# Autodesk Inventor assembly: Assembly1
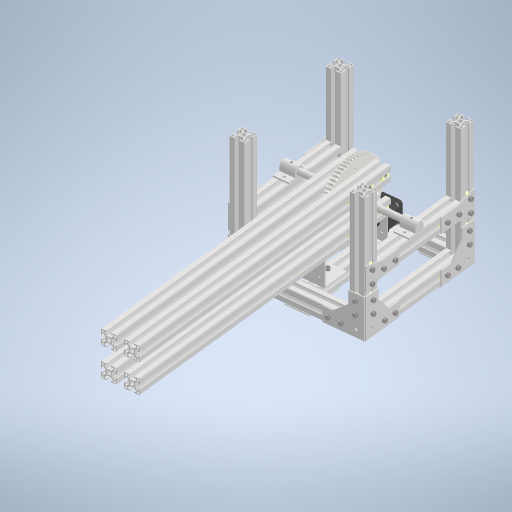
[picture p0: Inventor's stored thumbnail of the model, 512x512]
Saved by Autodesk Inventor 2024 (Build 280153000, 153)
## iProperties
Created: 2025-12-08
Part Number: Assembly1
Document SubType Name: Assembly
Designer: schar
Author: schar
## Documents named in this file (22)
- C:\Users\schar\Desktop\projectBlueprint\AMSTS\hardware\Assembly1.iam
- C:\Users\schar\Desktop\projectBlueprint\AMSTS\hardware\3030_200.ipt
- C:\Users\schar\Desktop\projectBlueprint\AMSTS\hardware\Connect2x3030_m6.ipt
- C:\Users\schar\Desktop\projectBlueprint\AMSTS\hardware\3030_tnut_m6.ipt
- C:\Users\schar\Documents\Inventor\Content Center Files\R2024\en-US\AS 1420\AS 1420 - 1973 - M5 x 10.ipt
- C:\Users\schar\Desktop\projectBlueprint\AMSTS\hardware\3030_260.ipt
- C:\Users\schar\Desktop\projectBlueprint\AMSTS\hardware\3030_connector_assembled.iam
- C:\Users\schar\Desktop\projectBlueprint\AMSTS\hardware\3030_connector_assembled_MIR.iam
- C:\Users\schar\Desktop\projectBlueprint\AMSTS\hardware\3030_connector_assembled_MIR1.iam
- C:\Users\schar\Desktop\projectBlueprint\AMSTS\hardware\3030_connector_assembled_MIR_MIR.iam
- C:\Users\schar\Desktop\projectBlueprint\AMSTS\hardware\3030_T_connector_assembled.iam
- C:\Users\schar\Desktop\projectBlueprint\AMSTS\hardware\3030_T_connector_assembled_MIR1.iam
- C:\Users\schar\Desktop\projectBlueprint\AMSTS\hardware\NEMA 17 - MS17HD2.iam
- C:\Users\schar\Desktop\projectBlueprint\AMSTS\hardware\wormgear_pol_base.iam
- C:\Users\schar\Desktop\projectBlueprint\AMSTS\hardware\base_axis_static_12mm.ipt
- C:\Users\schar\Desktop\projectBlueprint\AMSTS\hardware\base_axis_12mm.ipt
- C:\Users\schar\Desktop\projectBlueprint\AMSTS\hardware\NEMA17-3030-m6-holder.ipt
- C:\Users\schar\Desktop\projectBlueprint\AMSTS\hardware\3030_tnut_m6_main.ipt
- C:\Users\schar\Desktop\projectBlueprint\AMSTS\hardware\basis-bearing-3030-m6-holder.ipt
- C:\Users\schar\Desktop\projectBlueprint\AMSTS\hardware\wormgear_axis_6mm.ipt
- C:\Users\schar\Desktop\projectBlueprint\AMSTS\hardware\wormgear_worm_axes_holder.ipt
- C:\Users\schar\Desktop\projectBlueprint\AMSTS\hardware\Az_rot_3030_with_holes.ipt
## Components (94 placed, 21 different names)
1. 3030_tnut_m6_main:1 — Rotational:16
2. 3030_tnut_m6_main:2 — Rigid:3
3. 3030_tnut_m6_main:3 — Rotational:17, Flush:34
4. 3030_tnut_m6_main:4 — Rotational:18
5. wormgear_axis_6mm:1 — Mate:61, Mate:62, Mate:63, Mate:64, Mate:65
6. wormgear_worm_axes_holder:1 — Mate:64, Mate:65
7. Az_rot_3030_with_holes:1 — Mate:66, Mate:67, Mate:68, Mate:84, Mate:85, Mate:86, Mate:87, Mate:88, Mate:89
8. Az_rot_3030_with_holes:2 — Mate:75, Mate:76, Mate:77, Mate:90, Mate:91, Mate:92, Mate:93, Mate:94, Mate:95
9. Az_rot_3030_with_holes:3 — Mate:69, Mate:70, Mate:71, Mate:78, Mate:79, Mate:80, Mate:81, Mate:82, Mate:83
10. Az_rot_3030_with_holes:4 — Mate:72, Mate:73, Mate:74, Mate:96, Mate:97, Mate:98, Mate:99, Mate:100, Mate:101
11. 3030_tnut_m6_main:5 — Mate:80, Mate:81
12. 3030_tnut_m6_main:6 — Mate:82, Mate:83
13. 3030_tnut_m6_main:7 — Mate:84, Mate:87
14. 3030_tnut_m6_main:8 — Mate:78, Mate:79
15. 3030_tnut_m6_main:9 — Mate:85, Mate:88
16. 3030_tnut_m6_main:10 — Mate:86, Mate:89
17. 3030_tnut_m6_main:11 — Mate:96, Mate:97
18. 3030_tnut_m6_main:12 — Mate:99, Mate:101
19. 3030_tnut_m6_main:13 — Mate:98, Mate:100
20. 3030_tnut_m6_main:14 — Mate:90, Mate:92
21. 3030_tnut_m6_main:15 — Mate:91, Mate:93
22. 3030_tnut_m6_main:16 — Mate:94, Mate:95
23. 3030_200:1 — Mate:1, Mate:2, Flush:1, Flush:2, Mate:4, Flush:5, Flush:6, Symmetry:1, Mate:30, Mate:45, Flush:18, Mate:48
24. 3030_200:2 — Mate:3, Flush:3, Flush:4, Mate:6, Flush:9, Flush:10, Symmetry:2
25. Connect2x3030_m6:1 — Mate:1, Mate:2, Flush:1, Flush:2, Mate:3, Flush:3, Flush:4, Rigid:1, Rotational:5, Rotational:6, Rotational:7, Insert:11, Insert:12, Insert:14, Insert:15, Mate:19, Mate:20, Mate:21, Mate:36, Mate:37
26. Connect2x3030_m6:2 — Mate:4, Flush:5, Flush:6, Mate:5, Flush:7, Flush:8, Rotational:1, Rotational:2, Rotational:3, Rotational:4, Insert:6, Insert:7, Insert:9, Insert:10, Mate:10, Mate:11, Mate:12, Mate:32, Mate:33
27. Connect2x3030_m6:3 — Mate:8, Flush:11, Flush:12, Rotational:12, Rotational:13, Rotational:14, Rotational:15, Insert:1, Insert:2, Insert:4, Insert:5, Mate:13, Mate:14, Mate:15, Mate:40, Mate:41
28. Connect2x3030_m6:4 — Mate:6, Flush:9, Flush:10, Mate:7, Flush:13, Mate:9, Flush:14, Rotational:8, Rotational:9, Rotational:10, Rotational:11, Insert:16, Insert:17, Insert:18, Insert:20, Mate:16, Mate:17, Mate:18, Mate:23, Flush:15, Mate:25
29. 3030_200:3 — Mate:5, Flush:7, Flush:8, Mate:8, Flush:11, Flush:12, Symmetry:2, Mate:52
30. 3030_200:4 — Flush:13, Mate:9, Flush:14, Symmetry:1, Mate:53, Flush:23
31. 3030_connector_assembled:1 [sub-assembly] — Mate:24, Mate:25, Mate:26
32. 3030_connector_assembled:2 [sub-assembly] — Mate:22, Mate:23, Flush:15, Mate:26
33. 3030_connector_assembled_MIR:1 [sub-assembly] — Mate:27, Mate:39, Mate:40
34. 3030_connector_assembled_MIR:2 [sub-assembly] — Mate:27, Mate:38, Mate:41
35. 3030_connector_assembled_MIR1:1 [sub-assembly] — Mate:28, Mate:34, Mate:37
36. 3030_connector_assembled_MIR1:2 [sub-assembly] — Mate:28, Mate:35, Mate:36
37. 3030_connector_assembled_MIR_MIR:1 [sub-assembly] — Mate:29, Mate:30, Mate:33
38. 3030_connector_assembled_MIR_MIR:2 [sub-assembly] — Mate:29, Mate:31, Mate:32
39. 3030_260:1 — Mate:10, Mate:11, Mate:12, Mate:31, Mate:49, Flush:20
40. 3030_260:2 — Mate:13, Mate:14, Mate:15, Mate:38, Mate:39, Mate:42, Flush:16
41. 3030_260:3 — Mate:16, Mate:17, Mate:18, Mate:22, Mate:24, Mate:43, Flush:17
42. 3030_260:4 — Mate:19, Mate:20, Mate:21, Mate:34, Mate:35, Mate:50, Flush:21
43. NEMA 17 - MS17HD2:1 [sub-assembly] — Rotational:19, Rotational:20, Mate:61, Mate:62
44. wormgear_pol_base:1 [sub-assembly] — Rigid:2, Mate:63, Mate:66, Mate:67, Mate:68, Mate:69, Mate:70, Mate:71, Mate:72, Mate:73, Mate:74, Mate:75, Mate:76, Mate:77
45. base_axis_static_12mm:1 — Flush:30, Mate:57, Insert:22
46. base_axis_static_12mm:2 — Mate:58, Flush:31, Flush:32, Insert:21
47. base_axis_12mm:1 — Insert:21, Insert:22, Rigid:2
48. basis-bearing-3030-m6-holder:1 — Mate:60, Flush:35, Rotational:18, Flush:36, Rigid:3, Insert:23, Insert:24
49. NEMA17-3030-m6-holder:1 — Mate:59, Flush:33, Rotational:16, Rotational:17, Insert:25, Insert:26, Rotational:19, Rotational:20
50. 3030_T_connector_assembled:1 [sub-assembly] — Mate:43, Flush:17, Mate:56, Flush:29
51. 3030_T_connector_assembled:2 [sub-assembly] — Mate:42, Flush:16, Flush:26
52. 3030_T_connector_assembled_MIR1:1 [sub-assembly] — Mate:50, Flush:21, Mate:55, Flush:27, Flush:28
53. 3030_T_connector_assembled_MIR1:2 [sub-assembly] — Mate:49, Flush:20, Mate:54, Flush:24, Flush:25
54. 3030_T_connector_assembled:3 [sub-assembly] — Mate:45, Flush:18, Mate:47, Flush:19
55. 3030_200:5 — Mate:47, Mate:48, Flush:19, Mate:52, Flush:22, Mate:59, Flush:33, Flush:34, Mate:60, Flush:35, Flush:36
56. 3030_T_connector_assembled:4 [sub-assembly] — Mate:53, Flush:22, Flush:23
57. 3030_200:6 — Mate:55, Flush:27, Flush:28, Mate:56, Flush:29, Flush:30, Mate:57
58. 3030_200:7 — Mate:54, Flush:24, Flush:25, Flush:26, Mate:58, Flush:31, Flush:32
59. 3030_tnut_m6:1 — Rotational:12
60. 3030_tnut_m6:2 — Rotational:11
61. 3030_tnut_m6:3 — Rigid:1
62. 3030_tnut_m6:4 — Rotational:1
63. 3030_tnut_m6:5 — Rotational:13
64. 3030_tnut_m6:6 — Rotational:10
65. 3030_tnut_m6:7 — Rotational:5
66. 3030_tnut_m6:8 — Rotational:2
67. 3030_tnut_m6:9 — Rotational:15
68. 3030_tnut_m6:10 — Rotational:8
69. 3030_tnut_m6:11 — Rotational:6
70. 3030_tnut_m6:12 — Rotational:4
71. 3030_tnut_m6:13 — Rotational:14
72. 3030_tnut_m6:14 — Rotational:9
73. 3030_tnut_m6:15 — Rotational:7
74. 3030_tnut_m6:16 — Rotational:3
75. AS 1420 - Metric M5 x 10:1 — Insert:1
76. AS 1420 - Metric M5 x 10:2 — Insert:2
77. AS 1420 - Metric M5 x 10:4 — Insert:4
78. AS 1420 - Metric M5 x 10:5 — Insert:5
79. AS 1420 - Metric M5 x 10:6 — Insert:6
80. AS 1420 - Metric M5 x 10:7 — Insert:7
81. AS 1420 - Metric M5 x 10:9 — Insert:9
82. AS 1420 - Metric M5 x 10:10 — Insert:10
83. AS 1420 - Metric M5 x 10:11 — Insert:11
84. AS 1420 - Metric M5 x 10:12 — Insert:12
85. AS 1420 - Metric M5 x 10:14 — Insert:14
86. AS 1420 - Metric M5 x 10:15 — Insert:15
87. AS 1420 - Metric M5 x 10:16 — Insert:16
88. AS 1420 - Metric M5 x 10:17 — Insert:17
89. AS 1420 - Metric M5 x 10:18 — Insert:18
90. AS 1420 - Metric M5 x 10:20 — Insert:20
91. AS 1420 - Metric M5 x 10:21 — Insert:23
92. AS 1420 - Metric M5 x 10:22 — Insert:24
93. AS 1420 - Metric M5 x 10:23 — Insert:25
94. AS 1420 - Metric M5 x 10:24 — Insert:26
## Relationships (181: Mate 98, Flush 36, Insert 22, RevoluteJoint 20, WeldJoint 3, Symmetry 2)
- Mate:1: 3030_200:1 ↔ Connect2x3030_m6:1
- Mate:2: 3030_200:1 ↔ Connect2x3030_m6:1
- Flush:1: 3030_200:1 ↔ Connect2x3030_m6:1
- Flush:2 (30 mm): 3030_200:1 ↔ Connect2x3030_m6:1
- Mate:3: 3030_200:2 ↔ Connect2x3030_m6:1
- Flush:3 (30 mm): 3030_200:2 ↔ Connect2x3030_m6:1
- Flush:4: 3030_200:2 ↔ Connect2x3030_m6:1
- Mate:4: 3030_200:1 ↔ Connect2x3030_m6:2
- Flush:5 (-30 mm): 3030_200:1 ↔ Connect2x3030_m6:2
- Flush:6: 3030_200:1 ↔ Connect2x3030_m6:2
- Mate:5: Connect2x3030_m6:2 ↔ 3030_200:3
- Flush:7 (30 mm): Connect2x3030_m6:2 ↔ 3030_200:3
- Flush:8: Connect2x3030_m6:2 ↔ 3030_200:3
- Mate:6: 3030_200:2 ↔ Connect2x3030_m6:4
- Flush:9 (-30 mm): 3030_200:2 ↔ Connect2x3030_m6:4
- Flush:10: 3030_200:2 ↔ Connect2x3030_m6:4
- Mate:7: Connect2x3030_m6:4
- Mate:8: Connect2x3030_m6:3 ↔ 3030_200:3
- Flush:11 (-30 mm): Connect2x3030_m6:3 ↔ 3030_200:3
- Flush:12: Connect2x3030_m6:3 ↔ 3030_200:3
- Flush:13: Connect2x3030_m6:4 ↔ 3030_200:4
- Mate:9: Connect2x3030_m6:4 ↔ 3030_200:4
- Flush:14 (-30 mm): Connect2x3030_m6:4 ↔ 3030_200:4
- Rotational:1 [RevoluteJoint] (-0.357 mm): Connect2x3030_m6:2 ↔ 3030_tnut_m6:4
- Rotational:2 [RevoluteJoint] (-0.357 mm): Connect2x3030_m6:2 ↔ 3030_tnut_m6:8
- Rotational:3 [RevoluteJoint] (-0.357 mm): Connect2x3030_m6:2 ↔ 3030_tnut_m6:16
- Rotational:4 [RevoluteJoint] (-0.357 mm): Connect2x3030_m6:2 ↔ 3030_tnut_m6:12
- Rigid:1 [WeldJoint] (-0.357 mm): Connect2x3030_m6:1 ↔ 3030_tnut_m6:3
- Rotational:5 [RevoluteJoint] (-0.357 mm): Connect2x3030_m6:1 ↔ 3030_tnut_m6:7
- Rotational:6 [RevoluteJoint] (-0.357 mm): Connect2x3030_m6:1 ↔ 3030_tnut_m6:11
- Rotational:7 [RevoluteJoint] (-0.357 mm): Connect2x3030_m6:1 ↔ 3030_tnut_m6:15
- Rotational:8 [RevoluteJoint] (-0.357 mm): Connect2x3030_m6:4 ↔ 3030_tnut_m6:10
- Rotational:9 [RevoluteJoint] (-0.357 mm): Connect2x3030_m6:4 ↔ 3030_tnut_m6:14
- Rotational:10 [RevoluteJoint] (-0.357 mm): Connect2x3030_m6:4 ↔ 3030_tnut_m6:6
- Rotational:11 [RevoluteJoint] (-0.357 mm): Connect2x3030_m6:4 ↔ 3030_tnut_m6:2
- Rotational:12 [RevoluteJoint] (-0.357 mm): Connect2x3030_m6:3 ↔ 3030_tnut_m6:1
- Rotational:13 [RevoluteJoint]: Connect2x3030_m6:3 ↔ 3030_tnut_m6:5
- Rotational:14 [RevoluteJoint] (-0.357 mm): Connect2x3030_m6:3 ↔ 3030_tnut_m6:13
- Rotational:15 [RevoluteJoint] (-0.357 mm): Connect2x3030_m6:3 ↔ 3030_tnut_m6:9
- Insert:1: Connect2x3030_m6:3 ↔ AS 1420 - Metric M5 x 10:1
- Insert:2: Connect2x3030_m6:3 ↔ AS 1420 - Metric M5 x 10:2
- Insert:4: Connect2x3030_m6:3 ↔ AS 1420 - Metric M5 x 10:4
- Insert:5: Connect2x3030_m6:3 ↔ AS 1420 - Metric M5 x 10:5
- Insert:6: Connect2x3030_m6:2 ↔ AS 1420 - Metric M5 x 10:6
- Insert:7: Connect2x3030_m6:2 ↔ AS 1420 - Metric M5 x 10:7
- Insert:9: Connect2x3030_m6:2 ↔ AS 1420 - Metric M5 x 10:9
- Insert:10: Connect2x3030_m6:2 ↔ AS 1420 - Metric M5 x 10:10
- Insert:11: Connect2x3030_m6:1 ↔ AS 1420 - Metric M5 x 10:11
- Insert:12: Connect2x3030_m6:1 ↔ AS 1420 - Metric M5 x 10:12
- Insert:14: Connect2x3030_m6:1 ↔ AS 1420 - Metric M5 x 10:14
- Insert:15: Connect2x3030_m6:1 ↔ AS 1420 - Metric M5 x 10:15
- Insert:16: Connect2x3030_m6:4 ↔ AS 1420 - Metric M5 x 10:16
- Insert:17: Connect2x3030_m6:4 ↔ AS 1420 - Metric M5 x 10:17
- Insert:18: Connect2x3030_m6:4 ↔ AS 1420 - Metric M5 x 10:18
- Insert:20: Connect2x3030_m6:4 ↔ AS 1420 - Metric M5 x 10:20
- Mate:10: Connect2x3030_m6:2 ↔ 3030_260:1
- Mate:11: Connect2x3030_m6:2 ↔ 3030_260:1
- Mate:12: Connect2x3030_m6:2 ↔ 3030_260:1
- Mate:13: Connect2x3030_m6:3 ↔ 3030_260:2
- Mate:14: Connect2x3030_m6:3 ↔ 3030_260:2
- Mate:15: Connect2x3030_m6:3 ↔ 3030_260:2
- Mate:16: Connect2x3030_m6:4 ↔ 3030_260:3
- Mate:17: Connect2x3030_m6:4 ↔ 3030_260:3
- Mate:18: Connect2x3030_m6:4 ↔ 3030_260:3
- Mate:19: Connect2x3030_m6:1 ↔ 3030_260:4
- Mate:20: Connect2x3030_m6:1 ↔ 3030_260:4
- Mate:21: Connect2x3030_m6:1 ↔ 3030_260:4
- Symmetry:1: 3030_200:1 ↔ 3030_200:4
- Mate:22: 3030_connector_assembled:2 ↔ 3030_260:3
- Mate:23: Connect2x3030_m6:4 ↔ 3030_connector_assembled:2
- Flush:15: Connect2x3030_m6:4 ↔ 3030_connector_assembled:2
- Mate:24: 3030_connector_assembled:1 ↔ 3030_260:3
- Mate:25: Connect2x3030_m6:4 ↔ 3030_connector_assembled:1
- Mate:26: 3030_connector_assembled:1 ↔ 3030_connector_assembled:2
- Symmetry:2: 3030_200:2 ↔ 3030_200:3
- Mate:27: 3030_connector_assembled_MIR:1 ↔ 3030_connector_assembled_MIR:2
- Mate:28: 3030_connector_assembled_MIR1:1 ↔ 3030_connector_assembled_MIR1:2
- Mate:29: 3030_connector_assembled_MIR_MIR:1 ↔ 3030_connector_assembled_MIR_MIR:2
- Mate:30: 3030_200:1 ↔ 3030_connector_assembled_MIR_MIR:1
- Mate:31: 3030_connector_assembled_MIR_MIR:2 ↔ 3030_260:1
- Mate:32: Connect2x3030_m6:2 ↔ 3030_connector_assembled_MIR_MIR:2
- Mate:33: Connect2x3030_m6:2 ↔ 3030_connector_assembled_MIR_MIR:1
- Mate:34: 3030_connector_assembled_MIR1:1 ↔ 3030_260:4
- Mate:35: 3030_connector_assembled_MIR1:2 ↔ 3030_260:4
- Mate:36: Connect2x3030_m6:1 ↔ 3030_connector_assembled_MIR1:2
- Mate:37: Connect2x3030_m6:1 ↔ 3030_connector_assembled_MIR1:1
- Mate:38: 3030_connector_assembled_MIR:2 ↔ 3030_260:2
- Mate:39: 3030_connector_assembled_MIR:1 ↔ 3030_260:2
- Mate:40: Connect2x3030_m6:3 ↔ 3030_connector_assembled_MIR:1
- Mate:41: Connect2x3030_m6:3 ↔ 3030_connector_assembled_MIR:2
- Mate:42: 3030_260:2 ↔ 3030_T_connector_assembled:2
- Flush:16: 3030_260:2 ↔ 3030_T_connector_assembled:2
- Mate:43: 3030_260:3 ↔ 3030_T_connector_assembled:1
- Flush:17: 3030_260:3 ↔ 3030_T_connector_assembled:1
- Mate:45: 3030_200:1 ↔ 3030_T_connector_assembled:3
- Flush:18: 3030_200:1 ↔ 3030_T_connector_assembled:3
- Mate:47: 3030_T_connector_assembled:3 ↔ 3030_200:5
- Mate:48: 3030_200:1 ↔ 3030_200:5
- Flush:19: 3030_T_connector_assembled:3 ↔ 3030_200:5
- Mate:49: 3030_260:1 ↔ 3030_T_connector_assembled_MIR1:2
- Flush:20: 3030_260:1 ↔ 3030_T_connector_assembled_MIR1:2
- Mate:50: 3030_260:4 ↔ 3030_T_connector_assembled_MIR1:1
- Flush:21: 3030_260:4 ↔ 3030_T_connector_assembled_MIR1:1
- Mate:52 (85 mm): 3030_200:3 ↔ 3030_200:5
- Mate:53: 3030_200:4 ↔ 3030_T_connector_assembled:4
- Flush:22: 3030_200:5 ↔ 3030_T_connector_assembled:4
- Flush:23: 3030_200:4 ↔ 3030_T_connector_assembled:4
- Mate:54: 3030_T_connector_assembled_MIR1:2 ↔ 3030_200:7
- Flush:24: 3030_T_connector_assembled_MIR1:2 ↔ 3030_200:7
- Flush:25 (-30 mm): 3030_T_connector_assembled_MIR1:2 ↔ 3030_200:7
- Flush:26: 3030_T_connector_assembled:2 ↔ 3030_200:7
- Mate:55: 3030_T_connector_assembled_MIR1:1 ↔ 3030_200:6
- Flush:27: 3030_T_connector_assembled_MIR1:1 ↔ 3030_200:6
- Flush:28 (30 mm): 3030_T_connector_assembled_MIR1:1 ↔ 3030_200:6
- Mate:56: 3030_T_connector_assembled:1 ↔ 3030_200:6
- Flush:29: 3030_T_connector_assembled:1 ↔ 3030_200:6
- Flush:30: base_axis_static_12mm:1 ↔ 3030_200:6
- Mate:57: base_axis_static_12mm:1 ↔ 3030_200:6
- Mate:58: base_axis_static_12mm:2 ↔ 3030_200:7
- Flush:31: base_axis_static_12mm:2 ↔ 3030_200:7
- Flush:32 (-75 mm): base_axis_static_12mm:2 ↔ 3030_200:7
- Insert:21: base_axis_static_12mm:2 ↔ base_axis_12mm:1
- Insert:22: base_axis_static_12mm:1 ↔ base_axis_12mm:1
- Rigid:2 [WeldJoint] (5 mm): wormgear_pol_base:1 ↔ base_axis_12mm:1
- Mate:59: NEMA17-3030-m6-holder:1 ↔ 3030_200:5
- Flush:33 (-10 mm): NEMA17-3030-m6-holder:1 ↔ 3030_200:5
- Rotational:16 [RevoluteJoint] (-0.357 mm): 3030_tnut_m6_main:1 ↔ NEMA17-3030-m6-holder:1
- Rotational:17 [RevoluteJoint] (-0.357 mm): 3030_tnut_m6_main:3 ↔ NEMA17-3030-m6-holder:1
- Flush:34: 3030_tnut_m6_main:3 ↔ 3030_200:5
- Mate:60: basis-bearing-3030-m6-holder:1 ↔ 3030_200:5
- Flush:35 (5 mm): basis-bearing-3030-m6-holder:1 ↔ 3030_200:5
- Rotational:18 [RevoluteJoint] (-0.367 mm): 3030_tnut_m6_main:4 ↔ basis-bearing-3030-m6-holder:1
- Flush:36 (-10 mm): basis-bearing-3030-m6-holder:1 ↔ 3030_200:5
- Rigid:3 [WeldJoint] (-0.357 mm): 3030_tnut_m6_main:2 ↔ basis-bearing-3030-m6-holder:1
- Insert:23: basis-bearing-3030-m6-holder:1 ↔ AS 1420 - Metric M5 x 10:21
- Insert:24: basis-bearing-3030-m6-holder:1 ↔ AS 1420 - Metric M5 x 10:22
- Insert:25: NEMA17-3030-m6-holder:1 ↔ AS 1420 - Metric M5 x 10:23
- Insert:26: NEMA17-3030-m6-holder:1 ↔ AS 1420 - Metric M5 x 10:24
- Rotational:19 [RevoluteJoint]: NEMA 17 - MS17HD2:1 ↔ NEMA17-3030-m6-holder:1
- Rotational:20 [RevoluteJoint]: NEMA 17 - MS17HD2:1 ↔ NEMA17-3030-m6-holder:1
- Mate:61: wormgear_axis_6mm:1 ↔ NEMA 17 - MS17HD2:1
- Mate:62: wormgear_axis_6mm:1 ↔ NEMA 17 - MS17HD2:1
- Mate:63: wormgear_axis_6mm:1 ↔ wormgear_pol_base:1
- Mate:64: wormgear_axis_6mm:1 ↔ wormgear_worm_axes_holder:1
- Mate:65: wormgear_axis_6mm:1 ↔ wormgear_worm_axes_holder:1
- Mate:66: Az_rot_3030_with_holes:1 ↔ wormgear_pol_base:1
- Mate:67: Az_rot_3030_with_holes:1 ↔ wormgear_pol_base:1
- Mate:68: Az_rot_3030_with_holes:1 ↔ wormgear_pol_base:1
- Mate:69: Az_rot_3030_with_holes:3 ↔ wormgear_pol_base:1
- Mate:70: Az_rot_3030_with_holes:3 ↔ wormgear_pol_base:1
- Mate:71: Az_rot_3030_with_holes:3 ↔ wormgear_pol_base:1
- Mate:72: Az_rot_3030_with_holes:4 ↔ wormgear_pol_base:1
- Mate:73: Az_rot_3030_with_holes:4 ↔ wormgear_pol_base:1
- Mate:74: Az_rot_3030_with_holes:4 ↔ wormgear_pol_base:1
- Mate:75: Az_rot_3030_with_holes:2 ↔ wormgear_pol_base:1
- Mate:76: Az_rot_3030_with_holes:2 ↔ wormgear_pol_base:1
- Mate:77: Az_rot_3030_with_holes:2 ↔ wormgear_pol_base:1
- Mate:78: Az_rot_3030_with_holes:3 ↔ 3030_tnut_m6_main:8
- Mate:79: Az_rot_3030_with_holes:3 ↔ 3030_tnut_m6_main:8
- Mate:80: Az_rot_3030_with_holes:3 ↔ 3030_tnut_m6_main:5
- Mate:81: Az_rot_3030_with_holes:3 ↔ 3030_tnut_m6_main:5
- Mate:82: Az_rot_3030_with_holes:3 ↔ 3030_tnut_m6_main:6
- Mate:83: Az_rot_3030_with_holes:3 ↔ 3030_tnut_m6_main:6
- Mate:84: Az_rot_3030_with_holes:1 ↔ 3030_tnut_m6_main:7
- Mate:85: Az_rot_3030_with_holes:1 ↔ 3030_tnut_m6_main:9
- Mate:86: Az_rot_3030_with_holes:1 ↔ 3030_tnut_m6_main:10
- Mate:87: Az_rot_3030_with_holes:1 ↔ 3030_tnut_m6_main:7
- Mate:88: Az_rot_3030_with_holes:1 ↔ 3030_tnut_m6_main:9
- Mate:89: Az_rot_3030_with_holes:1 ↔ 3030_tnut_m6_main:10
- Mate:90: Az_rot_3030_with_holes:2 ↔ 3030_tnut_m6_main:14
- Mate:91: Az_rot_3030_with_holes:2 ↔ 3030_tnut_m6_main:15
- Mate:92: Az_rot_3030_with_holes:2 ↔ 3030_tnut_m6_main:14
- Mate:93: Az_rot_3030_with_holes:2 ↔ 3030_tnut_m6_main:15
- Mate:94: Az_rot_3030_with_holes:2 ↔ 3030_tnut_m6_main:16
- Mate:95: Az_rot_3030_with_holes:2 ↔ 3030_tnut_m6_main:16
- Mate:96: Az_rot_3030_with_holes:4 ↔ 3030_tnut_m6_main:11
- Mate:97: Az_rot_3030_with_holes:4 ↔ 3030_tnut_m6_main:11
- Mate:98: Az_rot_3030_with_holes:4 ↔ 3030_tnut_m6_main:13
- Mate:99: Az_rot_3030_with_holes:4 ↔ 3030_tnut_m6_main:12
- Mate:100: Az_rot_3030_with_holes:4 ↔ 3030_tnut_m6_main:13
- Mate:101: Az_rot_3030_with_holes:4 ↔ 3030_tnut_m6_main:12
